# Autodesk Inventor assembly: motor_block
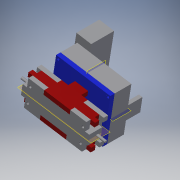
[picture p0: Inventor's stored thumbnail of the model, 180x180]
Saved by Autodesk Inventor 2019 (Build 230136000, 136)
## iProperties
Created: 2018-09-20
Part Number: motor_block
Material: Générique
Document SubType Name: Assembly
Designer: Jérémy
Author: Jérémy
## Documents named in this file (8)
- D:\Utilisateurs\Jérémy\Documents\Programmation\cubi\mechanics\motorbox\motor_block.iam
- D:\Utilisateurs\Jérémy\Documents\Programmation\cubi\mechanics\motorbox\moteur.ipt
- D:\Utilisateurs\Jérémy\Documents\Programmation\cubi\mechanics\motorbox\box.ipt
- D:\Utilisateurs\Jérémy\Documents\Programmation\cubi\mechanics\motorbox\board.ipt
- D:\Utilisateurs\Jérémy\Documents\Programmation\cubi\mechanics\motorbox\bat9V.ipt
- D:\Utilisateurs\Jérémy\Documents\Programmation\cubi\mechanics\motorbox\connector9V.ipt
- D:\Utilisateurs\Jérémy\Documents\Programmation\cubi\mechanics\motorbox\support_card.ipt
- D:\Utilisateurs\Jérémy\Documents\Programmation\cubi\mechanics\motorbox\cotes.xlsx
## Components (7 placed, 6 different names)
1. moteur:1 — Placage:1, Affleurement:1, Affleurement:2
2. moteur:2 — Placage:1, Affleurement:1, Affleurement:2, Affleurement:3, Affleurement:4
3. box:1 — Affleurement:3, Affleurement:4, Placage:2, Placage:3
4. board:1 — Logement:2, Affleurement:6
5. bat9V:1 — Logement:1, Affleurement:5
6. connector9V:1 — Logement:1, Affleurement:5, Logement:2
7. support_card:1 — Affleurement:6, Placage:2, Placage:3
## Relationships (11: Flush 6, Mate 3, Insert 2)
- Placage:1 [Mate] (20 mm): moteur:1 ↔ moteur:2
- Affleurement:1 [Flush]: moteur:1 ↔ moteur:2
- Affleurement:2 [Flush]: moteur:1 ↔ moteur:2
- Affleurement:3 [Flush]: moteur:2 ↔ box:1
- Affleurement:4 [Flush]: moteur:2 ↔ box:1
- Logement:1 [Insert]: bat9V:1 ↔ connector9V:1
- Affleurement:5 [Flush]: bat9V:1 ↔ connector9V:1
- Logement:2 [Insert]: board:1 ↔ connector9V:1
- Affleurement:6 [Flush]: board:1 ↔ support_card:1
- Placage:2 [Mate]: box:1 ↔ support_card:1
- Placage:3 [Mate]: box:1 ↔ support_card:1
## Named parameters: epaisseur = 5 mm, ecartement = 20 mm, dvis = 3 mm, largeur = 32 mm, L_fente = 30 mm, L_attache_carte = 15 mm, marge_attache_carte = 5 mm, L_cubi = 76.6 mm, largeur_cubi = 76.6 mm, taille_trou = 7 mm, L_moteur = 28.3 mm, marge_trou = 2 mm
